# Autodesk Inventor assembly: TopRobot
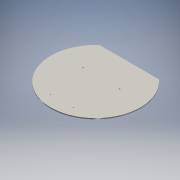
[picture p0: Inventor's stored thumbnail of the model, 180x180]
Saved by Autodesk Inventor 2019 (Build 230136000, 136)
## iProperties
Created: 2020-03-02
Part Number: TopRobot
Document SubType Name: Assembly
Designer: james
Author: james
## Documents named in this file (3)
- F:\JimsRobot\FIRSTRobots\Design\TornadoPlatypus\TopRobot.iam
- F:\JimsRobot\FIRSTRobots\Design\TornadoPlatypus\TopPlate.ipt
- F:\JimsRobot\FIRSTRobots\Design\Library\CTR\PDP_CAD\PDP_CAD_REV_1.0\3D\PDP_rev_1.0.ipt
## Components (2 placed, 2 different names)
1. TopPlate:1 — Mate:1, Mate:2, Mate:3
2. PDP_rev_1.0:1 — Mate:1, Mate:2, Mate:3
## Relationships (3: Mate 3)
- Mate:1: TopPlate:1 ↔ PDP_rev_1.0:1
- Mate:2: TopPlate:1 ↔ PDP_rev_1.0:1
- Mate:3: TopPlate:1 ↔ PDP_rev_1.0:1
